# Autodesk Inventor assembly: Overall_Assembly_Rev3
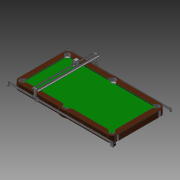
[picture p0: Inventor's stored thumbnail of the model, 180x180]
Saved by Autodesk Inventor 2015 (Build 190159000, 159)
## iProperties
Created: 2017-01-22
Part Number: Overall_Assembly_Rev3
Document SubType Name: Assembly
Designer: Guy
Author: Guy
## Documents named in this file (4)
- C:\Users\Guy\Documents\Fourth Year\Capstone\git\Capstone-Project\doc\CAD\LowLevel_Rev3\Overall_Assembly_Rev3.iam
- C:\Users\Guy\Documents\Fourth Year\Capstone\git\Capstone-Project\doc\CAD\Pool Table\Table_Model.ipt
- C:\Users\Guy\Documents\Fourth Year\Capstone\git\Capstone-Project\doc\CAD\LowLevel_Rev3\X_rail_Assembly_Rev3.iam
- C:\Users\Guy\Documents\Fourth Year\Capstone\git\Capstone-Project\doc\CAD\LowLevel_Rev3\Y_rail_Assembly_Rev3.iam
## Components (4 placed, 3 different names)
1. Table_Model:1 — Mate:1, Mate:2, Mate:3, Mate:4, Mate:5, Mate:6, Mate:7, Mate:8, Mate:9, Mate:10, Mate:11
2. X_rail_Assembly_Rev3:1 [sub-assembly] — Mate:1, Mate:2, Mate:3, Mate:4, Mate:5, Mate:6, Mate:7, Flush:1, Mate:12, Mate:13
3. X_rail_Assembly_Rev3:2 [sub-assembly] — Mate:8, Mate:9, Mate:10, Mate:11, Flush:1, Mate:14
4. Y_rail_Assembly_Rev3:1 [sub-assembly] — Mate:12, Mate:13, Mate:14
## Relationships (15: Mate 14, Flush 1)
- Mate:1 (40 mm): Table_Model:1 ↔ X_rail_Assembly_Rev3:1
- Mate:2: Table_Model:1 ↔ X_rail_Assembly_Rev3:1
- Mate:3: Table_Model:1 ↔ X_rail_Assembly_Rev3:1
- Mate:4: Table_Model:1 ↔ X_rail_Assembly_Rev3:1
- Mate:5: Table_Model:1 ↔ X_rail_Assembly_Rev3:1
- Mate:6: Table_Model:1 ↔ X_rail_Assembly_Rev3:1
- Mate:7: Table_Model:1 ↔ X_rail_Assembly_Rev3:1
- Mate:8: Table_Model:1 ↔ X_rail_Assembly_Rev3:2
- Mate:9: Table_Model:1 ↔ X_rail_Assembly_Rev3:2
- Mate:10 (40 mm): Table_Model:1 ↔ X_rail_Assembly_Rev3:2
- Mate:11: Table_Model:1 ↔ X_rail_Assembly_Rev3:2
- Flush:1: X_rail_Assembly_Rev3:1 ↔ X_rail_Assembly_Rev3:2
- Mate:12: X_rail_Assembly_Rev3:1 ↔ Y_rail_Assembly_Rev3:1
- Mate:13: X_rail_Assembly_Rev3:1 ↔ Y_rail_Assembly_Rev3:1
- Mate:14: X_rail_Assembly_Rev3:2 ↔ Y_rail_Assembly_Rev3:1
